# Autodesk Inventor assembly: cnc_2mm_v3
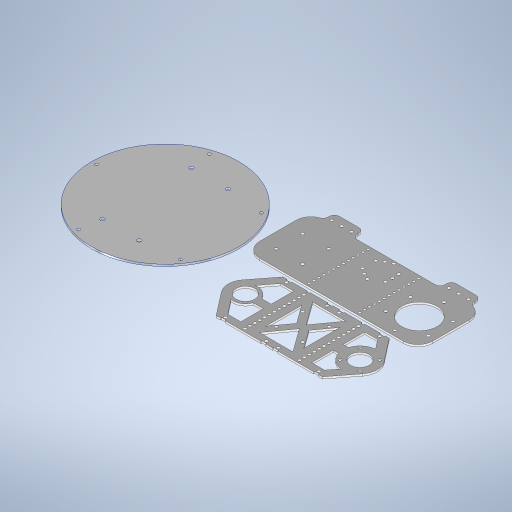
[picture p0: Inventor's stored thumbnail of the model, 512x512]
Saved by Autodesk Inventor 2024 (Build 280153000, 153)
## iProperties
Created: 2025-02-21
Part Number: cnc_2mm_v3
Document SubType Name: Assembly
Designer: tanoue_kota
Author: tanoue_kota
## Documents named in this file (4)
- C:\Users\田之上巧太\Documents\Inventor\RobArm\CNC\cnc_2mm_v3.iam
- C:\Users\田之上巧太\Documents\Inventor\RobArm\CNC\link1plate6\link1plate6.ipt
- C:\Users\田之上巧太\Documents\Inventor\RobArm\CNC\hand1_plate1\hand1_plate1.ipt
- C:\Users\田之上巧太\Documents\Inventor\RobArm\rob_base\base_plate7.ipt
## Components (3 placed, 3 different names)
1. link1plate6:1 — フラッシュ:1
2. hand1_plate1:1 — フラッシュ:1
3. base_plate7:1
## Relationships (1: Flush 1)
- フラッシュ:1 [Flush]: link1plate6:1 ↔ hand1_plate1:1
